# Autodesk Inventor assembly: CornerConnectAssyLeft
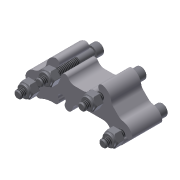
[picture p0: Inventor's stored thumbnail of the model, 180x180]
Saved by Autodesk Inventor 2013 (Build 170138000, 138)
## iProperties
Created: 2012-01-09
Part Number: CornerConnectAssyLeft
Document SubType Name: Assembly
Designer: Nemo
Author: Nemo
## Documents named in this file (4)
- \\lmss\STUDENTS\Robotics\CAD Files\COTS Parts\Kit Frame - AndyMark\Components\CornerConnectAssyRight.iam
- \\lmss\STUDENTS\Robotics\CAD Files\COTS Parts\Fasteners\14-20 locknut.ipt
- \\lmss\STUDENTS\Robotics\CAD Files\COTS Parts\Kit Frame - AndyMark\Components\Chassis Corner Connect.ipt
- \\lmss\STUDENTS\Robotics\CAD Files\COTS Parts\Fasteners\14-20 SHCS x1750.ipt
## Components (9 placed, 3 different names)
1. Chassis Corner Connect:1 — Insert:1, Insert:2, Insert:6, Insert:7, Insert:8, Insert:9, Insert:10, Insert:11
2. Hexagon Socket Head Cap Screw - Inch 1/4 - 20 UNC - 1 3/4:1 — Insert:1
3. 14-20 locknut:1 — Insert:2
4. Hexagon Socket Head Cap Screw - Inch 1/4 - 20 UNC - 1 3/4:2 — Insert:11
5. 14-20 locknut:2 — Insert:6
6. Hexagon Socket Head Cap Screw - Inch 1/4 - 20 UNC - 1 3/4:4 — Insert:7
7. 14-20 locknut:4 — Insert:8
8. Hexagon Socket Head Cap Screw - Inch 1/4 - 20 UNC - 1 3/4:5 — Insert:9
9. 14-20 locknut:5 — Insert:10
## Relationships (8: Insert 8)
- Insert:1 (3.175 mm): Chassis Corner Connect:1 ↔ Hexagon Socket Head Cap Screw - Inch 1/4 - 20 UNC - 1 3/4:1
- Insert:2 (3.302 mm): Chassis Corner Connect:1 ↔ 14-20 locknut:1
- Insert:6 (3.302 mm): Chassis Corner Connect:1 ↔ 14-20 locknut:2
- Insert:7 (3.175 mm): Chassis Corner Connect:1 ↔ Hexagon Socket Head Cap Screw - Inch 1/4 - 20 UNC - 1 3/4:4
- Insert:8 (3.302 mm): Chassis Corner Connect:1 ↔ 14-20 locknut:4
- Insert:9 (3.175 mm): Chassis Corner Connect:1 ↔ Hexagon Socket Head Cap Screw - Inch 1/4 - 20 UNC - 1 3/4:5
- Insert:10 (3.302 mm): Chassis Corner Connect:1 ↔ 14-20 locknut:5
- Insert:11 (3.175 mm): Chassis Corner Connect:1 ↔ Hexagon Socket Head Cap Screw - Inch 1/4 - 20 UNC - 1 3/4:2
